# Autodesk Inventor assembly: 2015 Summer Bevel Gearbox
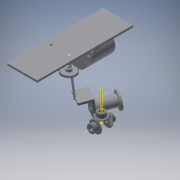
[picture p0: Inventor's stored thumbnail of the model, 180x180]
Saved by Autodesk Inventor 2016 (Build 200138000, 138)
## iProperties
Created: 2015-06-13
Part Number: 2015 Summer Bevel Gearbox
Document SubType Name: Assembly
Designer: steele
Author: steele
## Documents named in this file (14)
- C:\snobotics\CAD\robSteele\Bevel Gearbox\2015 Summer Bevel Gearbox.iam
- C:\snobotics\CAD\robSteele\Bevel Gearbox\2015 Summer Bevel Gearbox\Design Accelerator\Bevel Gears1.iam
- C:\snobotics\CAD\robSteele\Bevel Gearbox\2015 Summer Bevel Gearbox\Design Accelerator\Worm Gears1.iam
- C:\snobotics\CAD\robSteele\Bevel Gearbox\lift Hub.ipt
- C:\snobotics\CAD\robSteele\Bevel Gearbox\2015 Summer Bevel Gearbox\Angle Bracket for Bevel Gearbox.ipt
- C:\snobotics\CAD\robSteele\Bevel Gearbox\2015 Summer Bevel Gearbox\Design Accelerator\Bevel Gears1_MIR.iam
- C:\snobotics\CAD\partResources\BostonGear\wormAndWormGear\g1036.ipt
- C:\snobotics\CAD\partResources\BostonGear\wormAndWormGear\LUHB.ipt
- C:\snobotics\CAD\robSteele\ipart Components\0_250 in diam aluminum rod.ipt
- C:\snobotics\CAD\partResources\VexRobotics\Motors\Vex Mini Cim 217-3371.ipt
- C:\snobotics\CAD\partResources\Andy-Mark\motorMounts\AM 2488 CIM bracket.ipt
- C:\snobotics\CAD\robSteele\CIM to 0_1875 Worm Gearn.ipt
- C:\snobotics\CAD\robSteele\Bevel Gearbox\baseForWormMotor.ipt
- C:\snobotics\CAD\robSteele\ipart Components\0_250 in diam aluminum rod\0_250 in diam aluminum rod-02.ipt
## Components (12 placed, 12 different names)
1. Bevel Gears:1 [sub-assembly] — Angle:1
2. Worm Gears:1 [sub-assembly] — Angle:1
3. lift Hub:1 — Insert:5
4. Angle Bracket for Bevel Gearbox:1 — Mate:3, Mate:4, Mate:5, Insert:5, Tangent:1, Flush:7
5. Bevel Gears1_MIR:1 [sub-assembly]
6. g1036:1 — Insert:6
7. LUHB:1 — Insert:3
8. Vex Mini Cim 217-3371:1 — Insert:2, Insert:4
9. AM 2488 CIM bracket:1 — Insert:4, Mate:12, Flush:5, Flush:6
10. CIM to 0_1875 Worm Gearn:1 — Insert:2, Insert:3
11. baseForWormMotor:1 — Mate:12, Flush:5, Flush:6, Mate:14, Insert:6
12. 0_250 in diam aluminum rod-02:2 — Mate:14, Tangent:1, Flush:7
## Relationships (15: Mate 5, Insert 5, Flush 3, Angle 1, Tangent 1)
- Mate:3: Angle Bracket for Bevel Gearbox:1
- Mate:4: Angle Bracket for Bevel Gearbox:1
- Mate:5: Angle Bracket for Bevel Gearbox:1
- Insert:2: Vex Mini Cim 217-3371:1 ↔ CIM to 0_1875 Worm Gearn:1
- Insert:3: LUHB:1 ↔ CIM to 0_1875 Worm Gearn:1
- Insert:4: Vex Mini Cim 217-3371:1 ↔ AM 2488 CIM bracket:1
- Insert:5: lift Hub:1 ↔ Angle Bracket for Bevel Gearbox:1
- Mate:12: AM 2488 CIM bracket:1 ↔ baseForWormMotor:1
- Flush:5 (101.6 mm): AM 2488 CIM bracket:1 ↔ baseForWormMotor:1
- Flush:6: AM 2488 CIM bracket:1 ↔ baseForWormMotor:1
- Angle:1 (0 deg): Bevel Gears:1 ↔ Worm Gears:1
- Mate:14: baseForWormMotor:1 ↔ 0_250 in diam aluminum rod-02:2
- Insert:6 (28.6258 mm): g1036:1 ↔ baseForWormMotor:1
- Tangent:1: Angle Bracket for Bevel Gearbox:1 ↔ 0_250 in diam aluminum rod-02:2
- Flush:7: Angle Bracket for Bevel Gearbox:1 ↔ 0_250 in diam aluminum rod-02:2
